# Autodesk Inventor assembly: ArduinoUnoWithCase
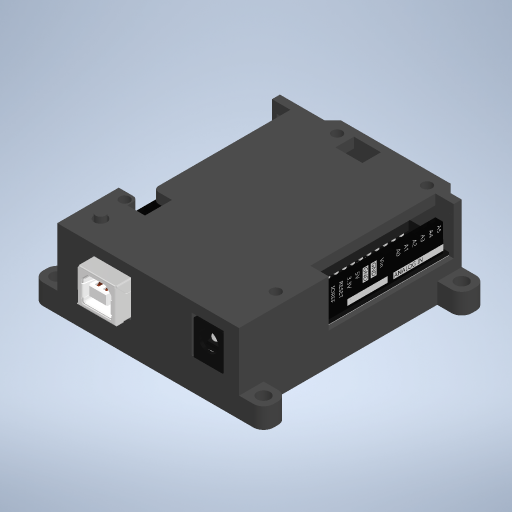
[picture p0: Inventor's stored thumbnail of the model, 512x512]
Saved by Autodesk Inventor 2024 (Build 280153000, 153)
## iProperties
Created: 2023-09-08
Part Number: ArduinoUnoWithCase
Document SubType Name: Assembly
Designer: 18179
Author: 18179
## Documents named in this file (5)
- C:\Users\18179\Desktop\TuppyMkIV_GitHub\TuppyMkIV\CAD\ArduinoUnoWithCase.iam
- C:\Users\18179\Desktop\TuppyMkIV_GitHub\TuppyMkIV\CAD\ArduinoCaseBottom.ipt
- C:\Users\18179\Desktop\TuppyMkIV_GitHub\TuppyMkIV\CAD\ArduinoCaseTop.ipt
- C:\Users\18179\Desktop\TuppyMkIV_GitHub\TuppyMkIV\CAD\Elegoo Uno R3.ipt
- C:\Users\18179\Desktop\TuppyMkIV_GitHub\TuppyMkIV\CAD\ArduinoCaseResetButton.ipt
## Components (4 placed, 4 different names)
1. ArduinoCaseBottom:1 — Mate:1, Mate:2, Mate:3, Mate:6
2. ArduinoCaseTop:1 — Mate:4, Mate:5, Mate:6
3. Elegoo Uno R3:1 — Mate:1, Mate:2, Mate:3, Mate:4, Mate:5, Mate:7, Mate:8
4. ArduinoCaseResetButton:1 — Mate:7, Mate:8
## Relationships (8: Mate 8)
- Mate:1: ArduinoCaseBottom:1 ↔ Elegoo Uno R3:1
- Mate:2: ArduinoCaseBottom:1 ↔ Elegoo Uno R3:1
- Mate:3: ArduinoCaseBottom:1 ↔ Elegoo Uno R3:1
- Mate:4: ArduinoCaseTop:1 ↔ Elegoo Uno R3:1
- Mate:5: ArduinoCaseTop:1 ↔ Elegoo Uno R3:1
- Mate:6: ArduinoCaseBottom:1 ↔ ArduinoCaseTop:1
- Mate:7: Elegoo Uno R3:1 ↔ ArduinoCaseResetButton:1
- Mate:8: Elegoo Uno R3:1 ↔ ArduinoCaseResetButton:1
